# Autodesk Inventor assembly: Hand ASM
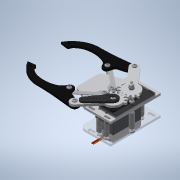
[picture p0: Inventor's stored thumbnail of the model, 180x180]
Saved by Autodesk Inventor 2020.3 (Build 243373000, 373)
## iProperties
Created: 2017-03-27
Part Number: Hand ASM
Document SubType Name: Assembly
Designer: Nanjar
Author: Nanjar
## Documents named in this file (18)
- C:\Users\Public\D\Desktop\robotic-arm-with-sensor-1.snapshot.1\Autodesk Inventor\_Robotic Arm With Sensor.iam
- C:\Users\Public\D\Desktop\robotic-arm-with-sensor-1.snapshot.1\Autodesk Inventor\TOWER PRO MG-995, ANALOG SERVO.iam
- C:\Users\Public\D\Desktop\robotic-arm-with-sensor-1.snapshot.1\Autodesk Inventor\ser Horn.ipt
- C:\Users\Public\D\Desktop\robotic-arm-with-sensor-1.snapshot.1\Autodesk Inventor\gearb2a.ipt
- C:\Users\Public\D\Desktop\robotic-arm-with-sensor-1.snapshot.1\Autodesk Inventor\arm1b.ipt
- C:\Users\Public\D\Desktop\robotic-arm-with-sensor-1.snapshot.1\Autodesk Inventor\claw2.ipt
- C:\Users\Public\D\Desktop\robotic-arm-with-sensor-1.snapshot.1\Autodesk Inventor\gearb2b.ipt
- C:\Users\Public\D\Desktop\robotic-arm-with-sensor-1.snapshot.1\Autodesk Inventor\spacer 6mm.ipt
- C:\Users\Public\D\Desktop\robotic-arm-with-sensor-1.snapshot.1\Autodesk Inventor\spacer 10mm.ipt
- C:\Users\Public\D\Desktop\robotic-arm-with-sensor-1.snapshot.1\Autodesk Inventor\Nut90591A121.ipt
- C:\Users\Public\D\Desktop\robotic-arm-with-sensor-1.snapshot.1\Autodesk Inventor\Dock bot2.ipt
- C:\Users\Public\D\Desktop\robotic-arm-with-sensor-1.snapshot.1\Autodesk Inventor\14Screw92005A124.ipt
- C:\Users\Public\D\Desktop\robotic-arm-with-sensor-1.snapshot.1\Autodesk Inventor\LNut90576A102.ipt
- C:\Users\Public\D\Desktop\robotic-arm-with-sensor-1.snapshot.1\Autodesk Inventor\10Screw92005A120.ipt
- C:\Users\Public\D\Desktop\robotic-arm-with-sensor-1.snapshot.1\Autodesk Inventor\20Screw92005A128.ipt
- C:\Users\Public\D\Desktop\robotic-arm-with-sensor-1.snapshot.1\Autodesk Inventor\Dock bot1 V2.ipt
- C:\Users\Public\D\Desktop\robotic-arm-with-sensor-1.snapshot.1\Autodesk Inventor\spacer 19mm.ipt
- C:\Users\Public\D\Desktop\robotic-arm-with-sensor-1.snapshot.1\Autodesk Inventor\Dock top2 V2.ipt
## Components (49 placed, 17 different names)
1. TOWER PRO MG-995, ANALOG SERVO:1 [sub-assembly] — Mate:1, Mate:2, Mate:7, Mate:80, Mate:112, Mate:113, Mate:171, Mate:172, Mate:173, Mate:174, Mate:177, Mate:178, Mate:179, Mate:180, Mate:183, Mate:184, Mate:185, Mate:186, Mate:193, Mate:194, Mate:196
2. ser Horn:1 — Mate:1, Mate:2, Mate:6, Mate:8, Mate:81
3. gearb2a:1 — Mate:6, Mate:7, Mate:8, Flush:1, Mate:13, Flush:2, Mate:14, Mate:15, Mate:17, Mate:31, Rotation:1, Angle:1, Mate:93, Mate:94
4. arm1b:1 — Mate:30, Mate:33, Mate:44, Mate:51, Mate:107
5. arm1b:2 — Mate:12, Mate:32, Mate:45, Mate:53
6. claw2:1 — Mate:29, Mate:30, Mate:33, Mate:99, Mate:100
7. claw2:2 — Mate:12, Mate:31, Mate:32, Mate:97, Mate:98
8. gearb2b:1 — Flush:1, Mate:16, Mate:17, Mate:29, Rotation:1, Mate:69, Mate:72, Mate:79, Mate:95, Mate:96
9. Dock bot2:1 — Mate:44, Mate:45, Mate:51, Mate:53, Mate:107, Mate:110, Mate:111, Mate:299, Mate:300, Mate:301
10. 14Screw92005A124:1 — Mate:72, Mate:77, Mate:309
11. Nut90591A121:2 — Mate:69, Mate:78, Mate:79
12. LNut90576A102:1 — Mate:77, Mate:78
13. 10Screw92005A120:1 — Mate:80, Mate:81
14. Nut90591A121:3
15. 10Screw92005A120:5 — Mate:93, Mate:94
16. 10Screw92005A120:7 — Mate:95, Mate:96
17. 10Screw92005A120:8 — Mate:97, Mate:98
18. 10Screw92005A120:9 — Mate:99, Mate:100
19. 20Screw92005A128:1 — Mate:283, Mate:305, Mate:308
20. 20Screw92005A128:2 — Mate:110
21. 20Screw92005A128:3 — Mate:111, Mate:270
22. Dock bot1 V2:1 — Mate:112, Mate:113, Mate:189, Mate:190, Mate:191, Mate:192, Mate:197, Mate:198, Mate:199, Mate:200, Mate:271, Mate:272, Mate:273, Mate:274, Mate:276, Mate:278, Mate:280, Mate:282, Mate:284, Mate:286
23. 20Screw92005A128:4 — Mate:275, Mate:306, Mate:307
24. spacer 6mm:9 — Mate:169, Mate:170
25. spacer 10mm:13 — Mate:169, Mate:170, Mate:171, Mate:172
26. Nut90591A121:7 — Mate:173, Mate:174
27. spacer 6mm:10
28. spacer 10mm:14 — Mate:179, Mate:180
29. Nut90591A121:8 — Mate:177, Mate:178
30. spacer 6mm:11
31. spacer 10mm:15 — Mate:183, Mate:184
32. Nut90591A121:9 — Mate:185, Mate:186
33. spacer 6mm:12
34. spacer 10mm:16 — Mate:193, Mate:194, Mate:195
35. Nut90591A121:10 — Mate:195, Mate:196
36. 10Screw92005A120:10 — Mate:189, Mate:190
37. 10Screw92005A120:11 — Mate:191, Mate:192
38. 10Screw92005A120:12 — Mate:197, Mate:200
39. 10Screw92005A120:13 — Mate:198, Mate:199
40. spacer 19mm:1 — Mate:270, Mate:271, Mate:272, Mate:279
41. spacer 19mm:2 — Mate:273, Mate:274, Mate:277
42. spacer 19mm:3 — Mate:275, Mate:276, Mate:281
43. Nut90591A121:20 — Mate:277, Mate:278
44. Nut90591A121:21 — Mate:279, Mate:280
45. Nut90591A121:22 — Mate:281, Mate:282
46. spacer 19mm:4 — Mate:283, Mate:284, Mate:285
47. Nut90591A121:23 — Mate:285, Mate:286
48. Dock top2 V2:1 — Mate:299, Mate:300, Mate:301, Mate:302, Mate:303, Mate:304
49. Dock top2 V2:2 — Mate:302, Mate:303, Mate:304, Mate:305, Mate:306, Mate:307, Mate:308, Mate:309
## Relationships (104: Mate 100, Flush 2, RelateRotation 1, Angle 1)
- Mate:1: TOWER PRO MG-995, ANALOG SERVO:1 ↔ ser Horn:1
- Mate:2: TOWER PRO MG-995, ANALOG SERVO:1 ↔ ser Horn:1
- Mate:6: ser Horn:1 ↔ gearb2a:1
- Mate:7: TOWER PRO MG-995, ANALOG SERVO:1 ↔ gearb2a:1
- Mate:8: ser Horn:1 ↔ gearb2a:1
- Mate:12: arm1b:2 ↔ claw2:2
- Flush:1: gearb2a:1 ↔ gearb2b:1
- Mate:13: gearb2a:1
- Flush:2: gearb2a:1
- Mate:14: gearb2a:1
- Mate:15: gearb2a:1
- Mate:16: gearb2b:1
- Mate:17 (26.23 mm): gearb2a:1 ↔ gearb2b:1
- Mate:29: claw2:1 ↔ gearb2b:1
- Mate:30: arm1b:1 ↔ claw2:1
- Mate:31: gearb2a:1 ↔ claw2:2
- Mate:32: arm1b:2 ↔ claw2:2
- Mate:33: arm1b:1 ↔ claw2:1
- Rotation:1 [RelateRotation] (1 ul): gearb2a:1 ↔ gearb2b:1
- Mate:44: arm1b:1 ↔ Dock bot2:1
- Mate:45: arm1b:2 ↔ Dock bot2:1
- Mate:51: arm1b:1 ↔ Dock bot2:1
- Mate:53: arm1b:2 ↔ Dock bot2:1
- Angle:1 (130.5 deg): gearb2a:1
- Mate:69: gearb2b:1 ↔ Nut90591A121:2
- Mate:72: gearb2b:1 ↔ 14Screw92005A124:1
- Mate:77: 14Screw92005A124:1 ↔ LNut90576A102:1
- Mate:78: Nut90591A121:2 ↔ LNut90576A102:1
- Mate:79: gearb2b:1 ↔ Nut90591A121:2
- Mate:80: TOWER PRO MG-995, ANALOG SERVO:1 ↔ 10Screw92005A120:1
- Mate:81: ser Horn:1 ↔ 10Screw92005A120:1
- Mate:93: gearb2a:1 ↔ 10Screw92005A120:5
- Mate:94: gearb2a:1 ↔ 10Screw92005A120:5
- Mate:95: gearb2b:1 ↔ 10Screw92005A120:7
- Mate:96: gearb2b:1 ↔ 10Screw92005A120:7
- Mate:97: claw2:2 ↔ 10Screw92005A120:8
- Mate:98: claw2:2 ↔ 10Screw92005A120:8
- Mate:99: claw2:1 ↔ 10Screw92005A120:9
- Mate:100: claw2:1 ↔ 10Screw92005A120:9
- Mate:107: arm1b:1 ↔ Dock bot2:1
- Mate:110: Dock bot2:1 ↔ 20Screw92005A128:2
- Mate:111: Dock bot2:1 ↔ 20Screw92005A128:3
- Mate:112: TOWER PRO MG-995, ANALOG SERVO:1 ↔ Dock bot1 V2:1
- Mate:113: TOWER PRO MG-995, ANALOG SERVO:1 ↔ Dock bot1 V2:1
- Mate:169: spacer 6mm:9 ↔ spacer 10mm:13
- Mate:170 (0.4 mm): spacer 6mm:9 ↔ spacer 10mm:13
- Mate:171: TOWER PRO MG-995, ANALOG SERVO:1 ↔ spacer 10mm:13
- Mate:172: TOWER PRO MG-995, ANALOG SERVO:1 ↔ spacer 10mm:13
- Mate:173: TOWER PRO MG-995, ANALOG SERVO:1 ↔ Nut90591A121:7
- Mate:174: TOWER PRO MG-995, ANALOG SERVO:1 ↔ Nut90591A121:7
- [Mate]: spacer 6mm:10 ↔ spacer 10mm:14
- [Mate] (0.4 mm): spacer 6mm:10 ↔ spacer 10mm:14
- Mate:177: TOWER PRO MG-995, ANALOG SERVO:1 ↔ Nut90591A121:8
- Mate:178: TOWER PRO MG-995, ANALOG SERVO:1 ↔ Nut90591A121:8
- Mate:179: TOWER PRO MG-995, ANALOG SERVO:1 ↔ spacer 10mm:14
- Mate:180: TOWER PRO MG-995, ANALOG SERVO:1 ↔ spacer 10mm:14
- [Mate]: spacer 6mm:11 ↔ spacer 10mm:15
- [Mate] (0.4 mm): spacer 6mm:11 ↔ spacer 10mm:15
- Mate:183: TOWER PRO MG-995, ANALOG SERVO:1 ↔ spacer 10mm:15
- Mate:184: TOWER PRO MG-995, ANALOG SERVO:1 ↔ spacer 10mm:15
- Mate:185: TOWER PRO MG-995, ANALOG SERVO:1 ↔ Nut90591A121:9
- Mate:186: TOWER PRO MG-995, ANALOG SERVO:1 ↔ Nut90591A121:9
- [Mate]: spacer 6mm:12 ↔ spacer 10mm:16
- [Mate] (0.4 mm): spacer 6mm:12 ↔ spacer 10mm:16
- Mate:189: Dock bot1 V2:1 ↔ 10Screw92005A120:10
- Mate:190: Dock bot1 V2:1 ↔ 10Screw92005A120:10
- Mate:191: Dock bot1 V2:1 ↔ 10Screw92005A120:11
- Mate:192: Dock bot1 V2:1 ↔ 10Screw92005A120:11
- Mate:193: TOWER PRO MG-995, ANALOG SERVO:1 ↔ spacer 10mm:16
- Mate:194: TOWER PRO MG-995, ANALOG SERVO:1 ↔ spacer 10mm:16
- Mate:195: spacer 10mm:16 ↔ Nut90591A121:10
- Mate:196: TOWER PRO MG-995, ANALOG SERVO:1 ↔ Nut90591A121:10
- Mate:197: Dock bot1 V2:1 ↔ 10Screw92005A120:12
- Mate:198: Dock bot1 V2:1 ↔ 10Screw92005A120:13
- Mate:199: Dock bot1 V2:1 ↔ 10Screw92005A120:13
- Mate:200: Dock bot1 V2:1 ↔ 10Screw92005A120:12
- Mate:270: 20Screw92005A128:3 ↔ spacer 19mm:1
- Mate:271: Dock bot1 V2:1 ↔ spacer 19mm:1
- Mate:272: Dock bot1 V2:1 ↔ spacer 19mm:1
- Mate:273: Dock bot1 V2:1 ↔ spacer 19mm:2
- Mate:274: Dock bot1 V2:1 ↔ spacer 19mm:2
- Mate:275: 20Screw92005A128:4 ↔ spacer 19mm:3
- Mate:276: Dock bot1 V2:1 ↔ spacer 19mm:3
- Mate:277: spacer 19mm:2 ↔ Nut90591A121:20
- Mate:278: Dock bot1 V2:1 ↔ Nut90591A121:20
- Mate:279: spacer 19mm:1 ↔ Nut90591A121:21
- Mate:280: Dock bot1 V2:1 ↔ Nut90591A121:21
- Mate:281: spacer 19mm:3 ↔ Nut90591A121:22
- Mate:282: Dock bot1 V2:1 ↔ Nut90591A121:22
- Mate:283: 20Screw92005A128:1 ↔ spacer 19mm:4
- Mate:284: Dock bot1 V2:1 ↔ spacer 19mm:4
- Mate:285: spacer 19mm:4 ↔ Nut90591A121:23
- Mate:286: Dock bot1 V2:1 ↔ Nut90591A121:23
- Mate:299: Dock bot2:1 ↔ Dock top2 V2:1
- Mate:300: Dock bot2:1 ↔ Dock top2 V2:1
- Mate:301: Dock bot2:1 ↔ Dock top2 V2:1
- Mate:302: Dock top2 V2:1 ↔ Dock top2 V2:2
- Mate:303: Dock top2 V2:1 ↔ Dock top2 V2:2
- Mate:304: Dock top2 V2:1 ↔ Dock top2 V2:2
- Mate:305: 20Screw92005A128:1 ↔ Dock top2 V2:2
- Mate:306: 20Screw92005A128:4 ↔ Dock top2 V2:2
- Mate:307: 20Screw92005A128:4 ↔ Dock top2 V2:2
- Mate:308: 20Screw92005A128:1 ↔ Dock top2 V2:2
- Mate:309: 14Screw92005A124:1 ↔ Dock top2 V2:2
## Named parameters: d224_d218 = 0 mm, d225_d219 = 0.4 mm, d230_d218 = 0 mm, d231_d219 = 0.4 mm, d236_d218 = 0 mm, d237_d219 = 0.4 mm
